# Autodesk Inventor assembly: manual shifter
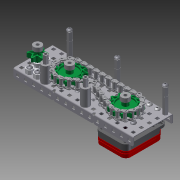
[picture p0: Inventor's stored thumbnail of the model, 180x180]
Saved by Autodesk Inventor 2014 SP1 (Build 180222100, 222)
## iProperties
Created: 2013-08-29
Part Number: manual shifter
Document SubType Name: Assembly
Designer: Ryan
Sending System: SolidWorks 2013
Last Author: Ryan
Author: Ryan
## Documents named in this file (20)
- C:\Users\Ryan\Desktop\sw\toss up 1st A bot\inventor drive\manual shifter.iam
- C:\Users\Ryan\Desktop\sw\lib\Aperture VEX CAD Library\Metal\C Channel\5 x 15.ipt
- C:\Users\Ryan\Desktop\sw\lib\Aperture VEX CAD Library\Bearing Blocks\Bearing Block.ipt
- C:\Users\Ryan\Desktop\sw\lib\Aperture VEX CAD Library\Hardware\8-32\8-32_.500.ipt
- C:\Users\Ryan\Desktop\sw\lib\Super Sonic Sparks VEX CAD Library\Motors & Sensors\Optical Shaft (Quadrature) Encoder.iam
- C:\Users\Ryan\Desktop\sw\lib\Aperture VEX CAD Library\Hardware\8-32\8-32_1.000.ipt
- C:\Users\Ryan\Desktop\sw\lib\Aperture VEX CAD Library\Spacers\SPACER-0500-0125.ipt
- C:\Users\Ryan\Desktop\sw\lib\Aperture VEX CAD Library\Hardware\Shaft Collar.ipt
- C:\Users\Ryan\Desktop\sw\lib\Aperture VEX CAD Library\Sprockets\green\High Strength 12-Tooth Sprocket.ipt
- C:\Users\Ryan\Desktop\sw\lib\Aperture VEX CAD Library\Spacers\spacer-0500-0500.ipt
- C:\Users\Ryan\Desktop\sw\lib\Aperture VEX CAD Library\Spacers\spacer-0500-0250.ipt
- C:\Users\Ryan\Desktop\sw\lib\Aperture VEX CAD Library\Sprockets\green\High Strength 6-Tooth Sprocket.ipt
- C:\Users\Ryan\Desktop\sw\lib\Aperture VEX CAD Library\Hardware\8-32\8-32 nylock.ipt
- C:\Users\Ryan\Desktop\sw\lib\Aperture VEX CAD Library\Standoffs\beam-0500.ipt
- C:\Users\Ryan\Desktop\sw\toss up 1st A bot\inventor drive\manual shifter\Design Accelerator\V-Belt transmission1.iam
- C:\Users\Ryan\Desktop\sw\lib\Aperture VEX CAD Library\Sprockets\HS Sprockets\High strength Chain Link.ipt
- C:\Users\Ryan\Desktop\sw\toss up 1st A bot\inventor drive\manual shifter\Design Accelerator\V-Belt transmission2.iam
- C:\Users\Ryan\Desktop\sw\lib\Aperture VEX CAD Library\Standoffs\BEAM-1000.ipt
- C:\Users\Ryan\Desktop\sw\lib\Aperture VEX CAD Library\Hardware\8-32\8-32_.375.ipt
- C:\Users\Ryan\Desktop\sw\lib\Aperture VEX CAD Library\Hardware\8-32\8-32_.875.ipt
## Components (122 placed, 22 different names)
1. 5 x 15:1 — Mate:1, Mate:2, Mate:3, Mate:4, Mate:7, Mate:8, Mate:9, Mate:12, Mate:13, Mate:14, Mate:15, Mate:16, Mate:17, Mate:18, Mate:23, Mate:24, Mate:26, Mate:28, Mate:42, Mate:43, Mate:44, Mate:47, Mate:54, Mate:62, Mate:63, Mate:66, Mate:67, Mate:68, Mate:69, Mate:72, Mate:73, Mate:74, Mate:76, Mate:94, Mate:95, Mate:98, Mate:99, Mate:103, Angle:1, Angle:2, Mate:113, Mate:114, Mate:115, Mate:120
2. V-Belt transmission:1 [sub-assembly]
3. V-Belt transmission:2 [sub-assembly]
4. spacer-0500-0125:1 — Mate:54, Mate:55, Mate:56, Mate:57
5. Shaft Collar:1 — Mate:56, Mate:57, Mate:58, Mate:59
6. 12 tooth hs sprocket:1 — Mate:58, Mate:59, Mate:60, Mate:61
7. spacer-0500-0250:1 — Mate:60, Mate:61
8. spacer-0500-0250:2 — Mate:52, Mate:53
9. Shaft Collar:2 — Mate:48, Mate:49, Mate:50, Mate:51
10. spacer-0500-0125:2 — Mate:46, Mate:47, Mate:48, Mate:49
11. 12 tooth hs sprocket:2 — Mate:50, Mate:51, Mate:52, Mate:53, Flush:1, Mate:109
12. 8-32_-500:11 — Mate:29, Mate:30, Mate:91
13. 8-32_-500:12 — Mate:25, Mate:27, Mate:92, Mate:96
14. bearing block:6 — Mate:23, Mate:24, Mate:25, Mate:26, Mate:27, Mate:28, Mate:29, Mate:30, Mate:31, Mate:32
15. 8-32 nylock:9 — Mate:91, Mate:94
16. 8-32 nylock:12 — Mate:92, Mate:96, Mate:98
17. spacer-0500-0125:5 — Mate:31, Mate:32, Mate:33, Mate:34
18. 6 tooth hs sprocket:1 — Mate:33, Mate:34, Mate:35, Mate:36, Mate:108
19. spacer-0500-0250:5 — Mate:35, Mate:36
20. bearing block:2 — Mate:1, Mate:2, Mate:3, Mate:4, Mate:5, Mate:6, Mate:83, Mate:85
21. 8-32_-500:3 — Mate:6, Mate:7, Mate:82
22. 8-32_-500:4 — Mate:5, Mate:8, Mate:84
23. 8-32 nylock:5 — Mate:82, Mate:83
24. 8-32 nylock:6 — Mate:84, Mate:85
25. bearing block:3 — Mate:9, Mate:10, Mate:11, Mate:12, Mate:13, Mate:14, Mate:46, Mate:88, Mate:89
26. 8-32_-500:5 — Mate:10, Mate:86
27. 8-32_-500:7 — Mate:11, Mate:87
28. 8-32 nylock:7 — Mate:86, Mate:89
29. 8-32 nylock:8 — Mate:87, Mate:88
30. bearing block:5 — Mate:15, Mate:16, Mate:17, Mate:18, Mate:20, Mate:37, Mate:38, Mate:39
31. 8-32_-500:9 — Mate:38, Mate:39, Mate:93, Mate:97
32. 8-32_-500:10 — Mate:20, Mate:37, Mate:90
33. 8-32 nylock:10 — Mate:90, Mate:95
34. 8-32 nylock:11 — Mate:93, Mate:97, Mate:99
35. bearing block:1 — Mate:55, Mate:62, Mate:63, Mate:64, Mate:65, Mate:66, Mate:67, Mate:81, Mate:106, Mate:107
36. 8-32_-500:1 — Mate:65, Mate:68, Mate:105
37. 8-32_-500:2 — Mate:64, Mate:69, Mate:104
38. 8-32 nylock:13 — Mate:105, Mate:106
39. 8-32 nylock:14 — Mate:104, Mate:107
40. OPTICAL-SHAFT-ENCODER:1 [sub-assembly] — Mate:71, Mate:77, Mate:79, Mate:81
41. beam-0500:6 — Mate:70
42. spacer-0500-0500:5 — Mate:40, Mate:41, Mate:43, Mate:70
43. spacer-0500-0500:4 — Mate:40, Mate:41, Mate:42, Mate:44, Mate:102
44. 8-32_.500:14 — Mate:102, Mate:103
45. BEAM-0500:10
46. SPACER-0500-0500:6
47. SPACER-0500-0500:7
48. 8-32_.500:15
49. High strength Chain Link:1 — Mate:108, Angle:1, Flush:1
50. High strength Chain Link:2
51. High strength Chain Link:3
52. High strength Chain Link:4
53. High strength Chain Link:5
54. High strength Chain Link:6
55. High strength Chain Link:7
56. High strength Chain Link:8
57. High strength Chain Link:9
58. High strength Chain Link:10
59. High strength Chain Link:11
60. High strength Chain Link:12
61. High strength Chain Link:13
62. High strength Chain Link:14
63. High strength Chain Link:15
64. High strength Chain Link:16
65. High strength Chain Link:17
66. High strength Chain Link:18
67. High strength Chain Link:19
68. High strength Chain Link:20
69. High strength Chain Link:21 — Mate:109, Angle:2
70. High strength Chain Link:22
71. High strength Chain Link:23
72. High strength Chain Link:24
73. High strength Chain Link:25
74. High strength Chain Link:26
75. High strength Chain Link:27
76. High strength Chain Link:28
77. High strength Chain Link:29
78. High strength Chain Link:30
79. High strength Chain Link:31
80. High strength Chain Link:32
81. High strength Chain Link:33
82. High strength Chain Link:34
83. High strength Chain Link:35
84. High strength Chain Link:36
85. High strength Chain Link:37
86. High strength Chain Link:38
87. High strength Chain Link:39
88. High strength Chain Link:40
89. High strength Chain Link:41
90. High strength Chain Link:42
91. High strength Chain Link:43
92. High strength Chain Link:44
93. High strength Chain Link:45
94. High strength Chain Link:46
95. High strength Chain Link:47
96. High strength Chain Link:48
97. High strength Chain Link:49
98. High strength Chain Link:50
99. High strength Chain Link:51
100. High strength Chain Link:52
101. High strength Chain Link:53
102. BEAM-1000:1 — Mate:115, Mate:116, Mate:119, Flush:2
103. BEAM-0500:11 — Mate:116, Mate:117, Mate:118, Mate:119, Flush:2
104. 8-32_.875:1 — Mate:117, Mate:118
105. 8-32_.375:1 — Mate:113, Mate:114, Mate:120
106. BEAM-1000:2
107. BEAM-0500:12
108. 8-32_.875:2
109. 8-32_.375:2
110. BEAM-1000:3
111. BEAM-0500:13
112. 8-32_.875:3
113. 8-32_.375:3
114. 8-32_1-000:2 — Mate:75, Mate:76, Mate:78, Mate:79
115. beam-0500:2 — Mate:71, Mate:72, Mate:73, Mate:74, Mate:75
116. 8-32 nylock:2 — Mate:77, Mate:78
117. 8-32_1.000:3
118. BEAM-0500:8
119. 8-32 nylock:15
120. 8-32_1.000:4
121. BEAM-0500:9
122. 8-32 nylock:16
## Component patterns: (2 elements, first: beam-0500:6 + spacer-0500-0500:5 + spacer-0500-0500:4 + 8-32_.500:14), (20 elements, first: High strength Chain Link:1), (33 elements, first: High strength Chain Link:21), (3 elements, first: BEAM-1000:1 + BEAM-0500:11 + 8-32_.875:1 + 8-32_.375:1), (3 elements, first: 8-32_1-000:2 + beam-0500:2 + 8-32 nylock:2)
## Relationships (116: Mate 112, Angle 2, Flush 2)
- Mate:1 (2.3114 mm): 5 x 15:1 ↔ bearing block:2
- Mate:2: 5 x 15:1 ↔ bearing block:2
- Mate:3 (2.3114 mm): 5 x 15:1 ↔ bearing block:2
- Mate:4 (2.3114 mm): 5 x 15:1 ↔ bearing block:2
- Mate:5: bearing block:2 ↔ 8-32_-500:4
- Mate:6: bearing block:2 ↔ 8-32_-500:3
- Mate:7: 5 x 15:1 ↔ 8-32_-500:3
- Mate:8: 5 x 15:1 ↔ 8-32_-500:4
- Mate:9: 5 x 15:1 ↔ bearing block:3
- Mate:10: bearing block:3 ↔ 8-32_-500:5
- Mate:11: bearing block:3 ↔ 8-32_-500:7
- Mate:12 (2.3114 mm): 5 x 15:1 ↔ bearing block:3
- Mate:13 (2.3114 mm): 5 x 15:1 ↔ bearing block:3
- Mate:14 (2.3114 mm): 5 x 15:1 ↔ bearing block:3
- Mate:15: 5 x 15:1 ↔ bearing block:5
- Mate:16 (2.3114 mm): 5 x 15:1 ↔ bearing block:5
- Mate:17 (2.3114 mm): 5 x 15:1 ↔ bearing block:5
- Mate:18 (2.3114 mm): 5 x 15:1 ↔ bearing block:5
- Mate:20: bearing block:5 ↔ 8-32_-500:10
- Mate:23: 5 x 15:1 ↔ bearing block:6
- Mate:24 (2.3114 mm): 5 x 15:1 ↔ bearing block:6
- Mate:25: 8-32_-500:12 ↔ bearing block:6
- Mate:26 (2.3114 mm): 5 x 15:1 ↔ bearing block:6
- Mate:27: 8-32_-500:12 ↔ bearing block:6
- Mate:28 (2.3114 mm): 5 x 15:1 ↔ bearing block:6
- Mate:29: 8-32_-500:11 ↔ bearing block:6
- Mate:30: 8-32_-500:11 ↔ bearing block:6
- Mate:31: bearing block:6 ↔ spacer-0500-0125:5
- Mate:32: bearing block:6 ↔ spacer-0500-0125:5
- Mate:33: spacer-0500-0125:5 ↔ 6 tooth hs sprocket:1
- Mate:34: spacer-0500-0125:5 ↔ 6 tooth hs sprocket:1
- Mate:35: 6 tooth hs sprocket:1 ↔ spacer-0500-0250:5
- Mate:36: 6 tooth hs sprocket:1 ↔ spacer-0500-0250:5
- Mate:37: bearing block:5 ↔ 8-32_-500:10
- Mate:38: bearing block:5 ↔ 8-32_-500:9
- Mate:39: bearing block:5 ↔ 8-32_-500:9
- Mate:40: spacer-0500-0500:5 ↔ spacer-0500-0500:4
- Mate:41: spacer-0500-0500:5 ↔ spacer-0500-0500:4
- Mate:42: 5 x 15:1 ↔ spacer-0500-0500:4
- Mate:43 (2.3114 mm): 5 x 15:1 ↔ spacer-0500-0500:5
- Mate:44 (2.3114 mm): 5 x 15:1 ↔ spacer-0500-0500:4
- [Mate]: beam-0500:6 ↔ spacer-0500-0500:5
- Mate:46: spacer-0500-0125:2 ↔ bearing block:3
- Mate:47: 5 x 15:1 ↔ spacer-0500-0125:2
- Mate:48: Shaft Collar:2 ↔ spacer-0500-0125:2
- Mate:49: Shaft Collar:2 ↔ spacer-0500-0125:2
- Mate:50: Shaft Collar:2 ↔ 12 tooth hs sprocket:2
- Mate:51: Shaft Collar:2 ↔ 12 tooth hs sprocket:2
- Mate:52: spacer-0500-0250:2 ↔ 12 tooth hs sprocket:2
- Mate:53: spacer-0500-0250:2 ↔ 12 tooth hs sprocket:2
- Mate:54: 5 x 15:1 ↔ spacer-0500-0125:1
- Mate:55: spacer-0500-0125:1 ↔ bearing block:1
- Mate:56: spacer-0500-0125:1 ↔ Shaft Collar:1
- Mate:57: spacer-0500-0125:1 ↔ Shaft Collar:1
- Mate:58: Shaft Collar:1 ↔ 12 tooth hs sprocket:1
- Mate:59: Shaft Collar:1 ↔ 12 tooth hs sprocket:1
- Mate:60: 12 tooth hs sprocket:1 ↔ spacer-0500-0250:1
- Mate:61: 12 tooth hs sprocket:1 ↔ spacer-0500-0250:1
- Mate:62 (2.3114 mm): 5 x 15:1 ↔ bearing block:1
- Mate:63: 5 x 15:1 ↔ bearing block:1
- Mate:64: bearing block:1 ↔ 8-32_-500:2
- Mate:65: bearing block:1 ↔ 8-32_-500:1
- Mate:66 (2.3114 mm): 5 x 15:1 ↔ bearing block:1
- Mate:67 (2.3114 mm): 5 x 15:1 ↔ bearing block:1
- Mate:68: 5 x 15:1 ↔ 8-32_-500:1
- Mate:69: 5 x 15:1 ↔ 8-32_-500:2
- Mate:70: beam-0500:6 ↔ spacer-0500-0500:5
- Mate:71: OPTICAL-SHAFT-ENCODER:1 ↔ beam-0500:2
- Mate:72 (2.3114 mm): 5 x 15:1 ↔ beam-0500:2
- Mate:73 (2.3114 mm): 5 x 15:1 ↔ beam-0500:2
- Mate:74: 5 x 15:1 ↔ beam-0500:2
- Mate:75: 8-32_1-000:2 ↔ beam-0500:2
- Mate:76: 5 x 15:1 ↔ 8-32_1-000:2
- Mate:77: OPTICAL-SHAFT-ENCODER:1 ↔ 8-32 nylock:2
- Mate:78: 8-32_1-000:2 ↔ 8-32 nylock:2
- Mate:79 (2.25 mm): OPTICAL-SHAFT-ENCODER:1 ↔ 8-32_1-000:2
- Mate:81: bearing block:1 ↔ OPTICAL-SHAFT-ENCODER:1
- Mate:82: 8-32_-500:3 ↔ 8-32 nylock:5
- Mate:83: bearing block:2 ↔ 8-32 nylock:5
- Mate:84: 8-32_-500:4 ↔ 8-32 nylock:6
- Mate:85: bearing block:2 ↔ 8-32 nylock:6
- Mate:86: 8-32_-500:5 ↔ 8-32 nylock:7
- Mate:87: 8-32_-500:7 ↔ 8-32 nylock:8
- Mate:88: bearing block:3 ↔ 8-32 nylock:8
- Mate:89: bearing block:3 ↔ 8-32 nylock:7
- Mate:90: 8-32_-500:10 ↔ 8-32 nylock:10
- Mate:91: 8-32_-500:11 ↔ 8-32 nylock:9
- Mate:92: 8-32_-500:12 ↔ 8-32 nylock:12
- Mate:93: 8-32_-500:9 ↔ 8-32 nylock:11
- Mate:94: 5 x 15:1 ↔ 8-32 nylock:9
- Mate:95: 5 x 15:1 ↔ 8-32 nylock:10
- Mate:96: 8-32_-500:12 ↔ 8-32 nylock:12
- Mate:97: 8-32_-500:9 ↔ 8-32 nylock:11
- Mate:98: 5 x 15:1 ↔ 8-32 nylock:12
- Mate:99: 5 x 15:1 ↔ 8-32 nylock:11
- Mate:102: spacer-0500-0500:4 ↔ 8-32_.500:14
- Mate:103: 5 x 15:1 ↔ 8-32_.500:14
- Mate:104: 8-32_-500:2 ↔ 8-32 nylock:14
- Mate:105: 8-32_-500:1 ↔ 8-32 nylock:13
- Mate:106: bearing block:1 ↔ 8-32 nylock:13
- Mate:107: bearing block:1 ↔ 8-32 nylock:14
- Mate:108: 6 tooth hs sprocket:1 ↔ High strength Chain Link:1
- Angle:1 (348.5 deg): 5 x 15:1 ↔ High strength Chain Link:1
- Flush:1: 12 tooth hs sprocket:2 ↔ High strength Chain Link:1
- Mate:109: 12 tooth hs sprocket:2 ↔ High strength Chain Link:21
- Angle:2 (32 deg): 5 x 15:1 ↔ High strength Chain Link:21
- [Mate]: BEAM-1000:1 ↔ 8-32_.375:1
- Mate:113: 5 x 15:1 ↔ 8-32_.375:1
- Mate:114 (2.3114 mm): 5 x 15:1 ↔ 8-32_.375:1
- Mate:115: 5 x 15:1 ↔ BEAM-1000:1
- Mate:116: BEAM-1000:1 ↔ BEAM-0500:11
- Mate:117: BEAM-0500:11 ↔ 8-32_.875:1
- Mate:118 (1.1684 mm): BEAM-0500:11 ↔ 8-32_.875:1
- Mate:119: BEAM-1000:1 ↔ BEAM-0500:11
- Flush:2: BEAM-1000:1 ↔ BEAM-0500:11
- Mate:120 (2.3114 mm): 5 x 15:1 ↔ 8-32_.375:1
## Named parameters: q = 2.3114 mm, encoder = 2.25 mm, d127_d51 = 0 mm, metal = 1.1684 mm
